# Autodesk Inventor assembly: Pump Mount Assembly
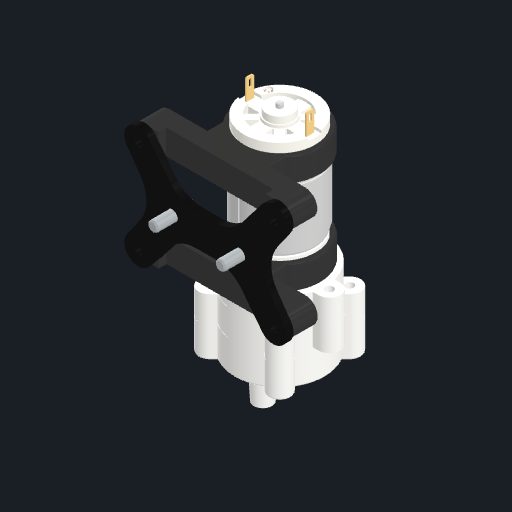
[picture p0: Inventor's stored thumbnail of the model, 512x512]
Saved by Autodesk Inventor 2024 (Build 280153000, 153)
## iProperties
Created: 2018-08-16
Part Number: Pump Mount Assembly
Document SubType Name: Assembly
Designer: Vincent Larson
Sending System: SolidWorks 2015
Last Author: Poseidon
Last Saved: 2018-08-17
Author: Vincent Larson
## Documents named in this file (3)
- C:\Users\Vincent Larson\Downloads\Pump Mount Assembly.iam
- C:\Users\Vincent Larson\Downloads\12v Pump.iam
- C:\Users\Vincent Larson\Downloads\Ender-3 Parts\01 MAIN ASM Ender_3\M3X6Pan Head Screw.ipt
## Components (5 placed, 2 different names)
1. 12v Pump:1 [sub-assembly] — Mate:2, Mate:3, Mate:4, Mate:5
2. M3X6Pan Head Screw:1 — Mate:4, Flush:1, Flush:2, Flush:3
3. M3X6Pan Head Screw:2 — Mate:2, Flush:2
4. M3X6Pan Head Screw:3 — Mate:5, Flush:1
5. M3X6Pan Head Screw:4 — Mate:3, Flush:3
## Relationships (7: Mate 4, Flush 3)
- Mate:2: 12v Pump:1 ↔ M3X6Pan Head Screw:2
- Mate:3: 12v Pump:1 ↔ M3X6Pan Head Screw:4
- Mate:4: 12v Pump:1 ↔ M3X6Pan Head Screw:1
- Mate:5: 12v Pump:1 ↔ M3X6Pan Head Screw:3
- Flush:1: M3X6Pan Head Screw:1 ↔ M3X6Pan Head Screw:3
- Flush:2: M3X6Pan Head Screw:1 ↔ M3X6Pan Head Screw:2
- Flush:3: M3X6Pan Head Screw:1 ↔ M3X6Pan Head Screw:4
